# Autodesk Inventor assembly: OUTER TORSO
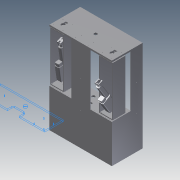
[picture p0: Inventor's stored thumbnail of the model, 180x180]
Saved by Autodesk Inventor 2011 (Build 150239000, 239)
## iProperties
Created: 2011-10-30
Part Number: OUTER TORSO
Document SubType Name: Assembly
Designer: Matthew
Author: Matthew
## Documents named in this file (7)
- C:\Users\Matthew\Documents\matthew_autocad\prlite\outer torso\OUTER TORSO.iam
- C:\Users\Matthew\Documents\matthew_autocad\prlite\outer torso\front.ipt
- C:\Users\Matthew\Documents\matthew_autocad\prlite\outer torso\holder.ipt
- C:\Users\Matthew\Documents\matthew_autocad\prlite\outer torso\side.ipt
- C:\Users\Matthew\Documents\matthew_autocad\prlite\outer torso\holdertop.ipt
- C:\Users\Matthew\Documents\matthew_autocad\prlite\arm perhaps\ARM SIMPLE 1.iam
- C:\Users\Matthew\Documents\matthew_autocad\prlite\arm perhaps\ARM SIMPLE 2.iam
## Components (7 placed, 6 different names)
1. front:1 — Mate:1, Mate:2, Flush:2, Flush:3, Mate:4, Flush:5, Flush:6, Flush:8, Flush:9, Mate:31
2. side:1 — Mate:1, Flush:3, Flush:8
3. side:2 — Mate:2, Flush:2, Flush:7, Flush:9, Flush:10
4. holder:1 — Mate:4, Flush:5, Flush:10, Mate:26, Mate:27, Mate:28, Mate:32, Mate:33, Mate:34
5. holdertop:1 — Flush:6, Flush:7, Mate:29, Mate:30, Mate:31, Mate:35
6. ARM SIMPLE 1:1 [sub-assembly] — Mate:26, Mate:27, Mate:28, Mate:29, Mate:30
7. ARM SIMPLE 2:1 [sub-assembly] — Mate:32, Mate:33, Mate:34, Mate:35
## Relationships (21: Mate 13, Flush 8)
- Mate:1: front:1 ↔ side:1
- Mate:2: front:1 ↔ side:2
- Flush:2: front:1 ↔ side:2
- Flush:3: front:1 ↔ side:1
- Mate:4: front:1 ↔ holder:1
- Flush:5: front:1 ↔ holder:1
- Flush:6: front:1 ↔ holdertop:1
- Flush:7: side:2 ↔ holdertop:1
- Flush:8: front:1 ↔ side:1
- Flush:9: front:1 ↔ side:2
- Flush:10: side:2 ↔ holder:1
- Mate:26: holder:1 ↔ ARM SIMPLE 1:1
- Mate:27: holder:1 ↔ ARM SIMPLE 1:1
- Mate:28: holder:1 ↔ ARM SIMPLE 1:1
- Mate:29: holdertop:1 ↔ ARM SIMPLE 1:1
- Mate:30: holdertop:1 ↔ ARM SIMPLE 1:1
- Mate:31: front:1 ↔ holdertop:1
- Mate:32: holder:1 ↔ ARM SIMPLE 2:1
- Mate:33: holder:1 ↔ ARM SIMPLE 2:1
- Mate:34: holder:1 ↔ ARM SIMPLE 2:1
- Mate:35: holdertop:1 ↔ ARM SIMPLE 2:1
